# Autodesk Inventor assembly: LegAssemblyLeftRear_MIR
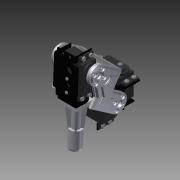
[picture p0: Inventor's stored thumbnail of the model, 180x180]
Saved by Autodesk Inventor 2015 (Build 190159000, 159)
## iProperties
Created: 2015-05-22
Part Number: LegAssemblyLeftRear_MIR
Document SubType Name: Assembly
Designer: Quinn
Author: Quinn
## Documents named in this file (8)
- C:\Users\Quinn\Documents\GitHub\Project-Onyx-Quadruped\Local-Only\3DCNC Design\InventorModels\Assemblies\LegAssemblyLeftRear_MIR.iam
- C:\Users\Quinn\Documents\GitHub\Project-Onyx-Quadruped\Local-Only\3DCNC Design\InventorModels\Assemblies\FXR_HipServo_MIR.iam
- C:\Users\Quinn\Documents\GitHub\Project-Onyx-Quadruped\Local-Only\3DCNC Design\InventorModels\Assemblies\Knee_LeftRear_MIR.iam
- C:\Users\Quinn\Documents\GitHub\Project-Onyx-Quadruped\Local-Only\3DCNC Design\InventorModels\Assemblies\FXL_HipServo_MIR.iam
- C:\Users\Quinn\Documents\GitHub\Project-Onyx-Quadruped\Local-Only\3DCNC Design\InventorModels\Assemblies\Foot_MIR.iam
- C:\Users\Quinn\Documents\GitHub\Project-Onyx-Quadruped\Local-Only\3DCNC Design\InventorModels\Assemblies\LegAssemblyLeftRear_MIR\Design Accelerator\Bolted Connection1.iam
- C:\Users\Quinn\Documents\GitHub\Project-Onyx-Quadruped\Local-Only\3DCNC Design\InventorModels\Assemblies\LegAssemblyLeftRear_MIR\Design Accelerator\Bolted Connection3.iam
- C:\Users\Quinn\Documents\GitHub\Project-Onyx-Quadruped\Local-Only\3DCNC Design\InventorModels\Assemblies\LegAssemblyLeftRear_MIR\Design Accelerator\Bolted Connection4.iam
## Components (8 placed, 5 different names)
1. FXR_HipServo_MIR:1 [sub-assembly] — Mate:1, Mate:9, Mate:10
2. FXR_HipServo_MIR:2 [sub-assembly] — Mate:1, Rotational:1
3. Knee_LeftRear_MIR:1 [sub-assembly] — Rotational:1, Rotational:2
4. FXL_HipServo_MIR:1 [sub-assembly] — Mate:6, Mate:5, Mate:4, Rotational:2
5. Foot_MIR:1 [sub-assembly] — Mate:6, Mate:5, Mate:4, Mate:11, Mate:12, Mate:13, Mate:14
6. Bolted Connection:1 [sub-assembly] — Mate:11, Mate:12
7. Bolted Connection:3 [sub-assembly] — Mate:9, Mate:10
8. Bolted Connection:4 [sub-assembly] — Mate:13, Mate:14
## Relationships (12: Mate 10, RevoluteJoint 2)
- Mate:1: FXR_HipServo_MIR:1 ↔ FXR_HipServo_MIR:2
- Mate:6: FXL_HipServo_MIR:1 ↔ Foot_MIR:1
- Mate:5: FXL_HipServo_MIR:1 ↔ Foot_MIR:1
- Mate:4: FXL_HipServo_MIR:1 ↔ Foot_MIR:1
- Rotational:1 [RevoluteJoint]: FXR_HipServo_MIR:2 ↔ Knee_LeftRear_MIR:1
- Rotational:2 [RevoluteJoint]: Knee_LeftRear_MIR:1 ↔ FXL_HipServo_MIR:1
- Mate:9: FXR_HipServo_MIR:1 ↔ Bolted Connection:3
- Mate:10: FXR_HipServo_MIR:1 ↔ Bolted Connection:3
- Mate:11: Foot_MIR:1 ↔ Bolted Connection:1
- Mate:12: Foot_MIR:1 ↔ Bolted Connection:1
- Mate:13: Foot_MIR:1 ↔ Bolted Connection:4
- Mate:14: Foot_MIR:1 ↔ Bolted Connection:4
